# Autodesk Inventor assembly: Fender and Igus_MIR1
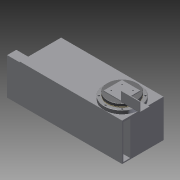
[picture p0: Inventor's stored thumbnail of the model, 180x180]
Saved by Autodesk Inventor 2015 (Build 190159000, 159)
## iProperties
Created: 2015-01-19
Part Number: Fender and Igus_MIR1
Document SubType Name: Assembly
Designer: chapale16
Author: chapale16
## Documents named in this file (5)
- \\lhssvr02\Homedirs\Robotics Club\CAD Model 2015\Fender and Igus_MIR1.iam
- \\lhssvr02\Homedirs\Robotics Club\CAD Model 2015\Bearing plate version 2.0_MIR1.ipt
- \\lhssvr02\Homedirs\Robotics Club\CAD Model 2015\Fc Fender Assembly_MIR2.iam
- \\lhssvr02\Homedirs\Robotics Club\CAD Model 2015\Igus and Arm Bracket_MIR.iam
- \\lhssvr02\Homedirs\Robotics Club\CAD Model 2015\Game Components\The Tote Collector-Arms\Tote Collector Arm_MIR_MIR.iam
## Components (4 placed, 4 different names)
1. Bearing plate version 2.0_MIR1:1 — Mate:5, Flush:2, Flush:1, Mate:3, Mate:6, Mate:4
2. Fc Fender Assembly_MIR2:1 [sub-assembly] — Mate:5, Flush:2, Flush:1, Mate:3
3. Igus and Arm Bracket_MIR:1 [sub-assembly] — Mate:6, Mate:4, Flush:3, Mate:8, Mate:7
4. Tote Collector Arm_MIR_MIR:1 [sub-assembly] — Flush:3, Mate:8, Mate:7
## Relationships (9: Mate 6, Flush 3)
- Mate:5: Bearing plate version 2.0_MIR1:1 ↔ Fc Fender Assembly_MIR2:1
- Flush:2: Bearing plate version 2.0_MIR1:1 ↔ Fc Fender Assembly_MIR2:1
- Flush:1: Bearing plate version 2.0_MIR1:1 ↔ Fc Fender Assembly_MIR2:1
- Mate:3: Bearing plate version 2.0_MIR1:1 ↔ Fc Fender Assembly_MIR2:1
- Mate:6: Bearing plate version 2.0_MIR1:1 ↔ Igus and Arm Bracket_MIR:1
- Mate:4: Bearing plate version 2.0_MIR1:1 ↔ Igus and Arm Bracket_MIR:1
- Flush:3: Igus and Arm Bracket_MIR:1 ↔ Tote Collector Arm_MIR_MIR:1
- Mate:8: Igus and Arm Bracket_MIR:1 ↔ Tote Collector Arm_MIR_MIR:1
- Mate:7: Igus and Arm Bracket_MIR:1 ↔ Tote Collector Arm_MIR_MIR:1
